# Autodesk Inventor assembly: Medium Tube + Medium Cap
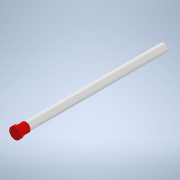
[picture p0: Inventor's stored thumbnail of the model, 180x180]
Saved by Autodesk Inventor 2020.1 (Build 241239000, 239)
## iProperties
Created: 2020-11-17
Part Number: Medium Tube + Medium Cap
Document SubType Name: Assembly
Designer: uqphoop1
Author: uqphoop1
## Documents named in this file (3)
- \\uq.edu.au\UQ-Inst-Gateway1\VALQSM2019-Q1896\Round phantoms\Vial and Cap Assembly\Medium Tube + Medium Cap.iam
- \\uq.edu.au\UQ-Inst-Gateway1\VALQSM2019-Q1896\Round phantoms\Medium tube_forMainAssembly.ipt
- \\uq.edu.au\UQ-Inst-Gateway1\VALQSM2019-Q1896\Round phantoms\10 mm Cap_forMainAssembly.ipt
## Components (2 placed, 2 different names)
1. Medium tube_forMainAssembly:1 — Insert:1
2. 10 mm Cap_forMainAssembly:1 — Insert:1
## Relationships (1: Insert 1)
- Insert:1: Medium tube_forMainAssembly:1 ↔ 10 mm Cap_forMainAssembly:1
